# Autodesk Inventor assembly: rf_tester
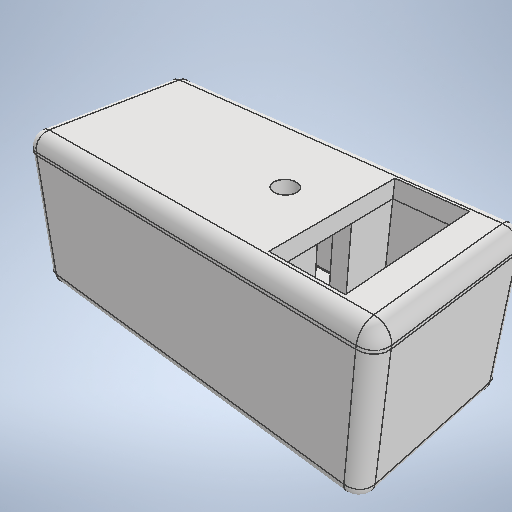
[picture p0: Inventor's stored thumbnail of the model, 512x512]
Saved by Autodesk Inventor 2025 (Build 290162000, 162)
## iProperties
Created: 2025-01-11
Part Number: rf_tester
Document SubType Name: Assembly
Designer: Jacob
Author: Jacob
## Documents named in this file (3)
- \\192.168.1.10\jake\Projects\XBOX_360\rf_tester\rf_tester.iam
- \\192.168.1.10\jake\Projects\XBOX_360\rf_tester\rf_tester_bottom.ipt
- \\192.168.1.10\jake\Projects\XBOX_360\rf_tester\rf_tester_top.ipt
## Components (2 placed, 2 different names)
1. rf_tester_bottom:1 — Flush:1, Flush:2, Flush:3, Flush:4
2. rf_tester_top:1 — Flush:1, Flush:2, Flush:3, Flush:4
## Relationships (4: Flush 4)
- Flush:1: rf_tester_bottom:1 ↔ rf_tester_top:1
- Flush:2: rf_tester_bottom:1 ↔ rf_tester_top:1
- Flush:3 (1.6 mm): rf_tester_bottom:1 ↔ rf_tester_top:1
- Flush:4: rf_tester_bottom:1 ↔ rf_tester_top:1
